# Autodesk Inventor assembly: El Cangrejo
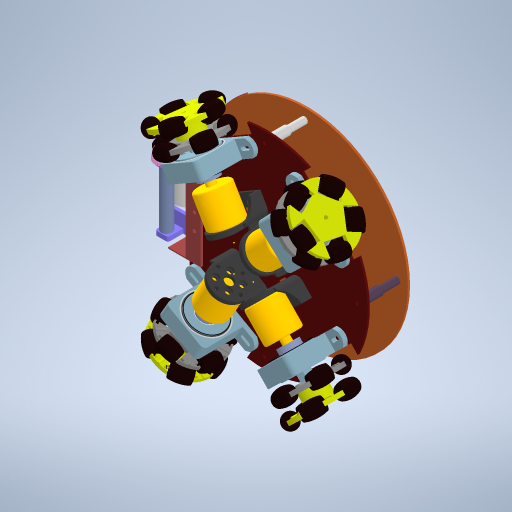
[picture p0: Inventor's stored thumbnail of the model, 512x512]
Saved by Autodesk Inventor 2024.2 (Build 282272000, 272)
## iProperties
Created: 2023-11-20
Part Number: El Cangrejo
Document SubType Name: Assembly
Designer: felip
Author: felip
## Documents named in this file (9)
- C:\Users\felip\Documentos\Robocupp-Mecanica\Gemelo Digital V2\El Cangrejo.iam
- C:\Users\felip\Documentos\Robocupp-Mecanica\Gemelo Digital V2\Motor-Soporte-Montaje.iam
- C:\Users\felip\Documentos\Robocupp-Mecanica\Gemelo Digital V2\Engranaje-Planetario-Montaje.iam
- C:\Users\felip\Documentos\Robocupp-Mecanica\Gemelo Digital V2\BaseV3-Piso2-Step.ipt
- C:\Users\felip\Documentos\Robocupp-Mecanica\Gemelo Digital V2\OMNIWHEELV4.iam
- C:\Users\felip\Documentos\Robocupp-Mecanica\Gemelo Digital V2\Pilar.ipt
- C:\Users\felip\Documentos\Robocupp-Mecanica\Gemelo Digital V2\Part Studio 1 - Part 1.ipt
- C:\Users\felip\Documentos\Robocupp-Mecanica\Gemelo Digital V2\Base-Dribler.ipt
- C:\Users\felip\Documentos\Robocupp-Mecanica\Gemelo Digital V2\Dribler-Desmontable.iam
## Components (19 placed, 8 different names)
1. Motor-Soporte-Montaje:1 [sub-assembly] — Rotational:5, Rotational:6, Cylindrical:4
2. Engranaje-Planetario-Montaje:1 [sub-assembly] — Cylindrical:3, Mate:3, Rotational:18
3. BaseV3-Piso2-Step:1 — Rotational:16, Rotational:17, Rotational:22, Rotational:23
4. OMNIWHEELV4:1 [sub-assembly] — Rotational:18
5. Pilar:1 — Rotational:13
6. Motor-Soporte-Montaje:2 [sub-assembly] — Rotational:7, Rotational:8, Cylindrical:2
7. Motor-Soporte-Montaje:3 [sub-assembly] — Rotational:3, Rotational:4, Cylindrical:1
8. Motor-Soporte-Montaje:4 [sub-assembly] — Rotational:1, Rotational:2, Cylindrical:3
9. Engranaje-Planetario-Montaje:2 [sub-assembly] — Cylindrical:1, Flush:1, Rotational:21
10. Engranaje-Planetario-Montaje:3 [sub-assembly] — Cylindrical:4, Flush:2, Rotational:20
11. Engranaje-Planetario-Montaje:4 [sub-assembly] — Cylindrical:2, Mate:1, Mate:2, Rotational:19
12. OMNIWHEELV4:2 [sub-assembly] — Rotational:19
13. OMNIWHEELV4:3 [sub-assembly] — Rotational:20
14. OMNIWHEELV4:4 [sub-assembly] — Rotational:21
15. Part Studio 1 - Part 1:1 — Rotational:1, Rotational:2, Rotational:3, Rotational:4, Rotational:5, Rotational:6, Rotational:7, Rotational:8, Flush:1, Mate:1, Mate:2, Mate:3, Flush:2, Rotational:13, Rotational:14, Rotational:15
16. Pilar:2 — Rotational:15, Rotational:17
17. Pilar:3 — Rotational:14, Rotational:16
18. Base-Dribler:1 — Rotational:22, Rotational:23, Planar:1, Planar:2
19. Dribler-Desmontable:1 [sub-assembly] — Planar:1, Planar:2
## Relationships (30: RevoluteJoint 19, CylindricalJoint 4, Mate 3, Flush 2, PlanarJoint 2)
- Rotational:1 [RevoluteJoint]: Motor-Soporte-Montaje:4 ↔ Part Studio 1 - Part 1:1
- Rotational:2 [RevoluteJoint]: Motor-Soporte-Montaje:4 ↔ Part Studio 1 - Part 1:1
- Rotational:3 [RevoluteJoint]: Motor-Soporte-Montaje:3 ↔ Part Studio 1 - Part 1:1
- Rotational:4 [RevoluteJoint]: Motor-Soporte-Montaje:3 ↔ Part Studio 1 - Part 1:1
- Rotational:5 [RevoluteJoint]: Motor-Soporte-Montaje:1 ↔ Part Studio 1 - Part 1:1
- Rotational:6 [RevoluteJoint]: Motor-Soporte-Montaje:1 ↔ Part Studio 1 - Part 1:1
- Rotational:7 [RevoluteJoint]: Motor-Soporte-Montaje:2 ↔ Part Studio 1 - Part 1:1
- Rotational:8 [RevoluteJoint]: Motor-Soporte-Montaje:2 ↔ Part Studio 1 - Part 1:1
- Cylindrical:1: Motor-Soporte-Montaje:3 ↔ Engranaje-Planetario-Montaje:2
- Flush:1: Engranaje-Planetario-Montaje:2 ↔ Part Studio 1 - Part 1:1
- Cylindrical:2: Motor-Soporte-Montaje:2 ↔ Engranaje-Planetario-Montaje:4
- Mate:1: Engranaje-Planetario-Montaje:4 ↔ Part Studio 1 - Part 1:1
- Mate:2: Engranaje-Planetario-Montaje:4 ↔ Part Studio 1 - Part 1:1
- Cylindrical:3: Engranaje-Planetario-Montaje:1 ↔ Motor-Soporte-Montaje:4
- Mate:3: Engranaje-Planetario-Montaje:1 ↔ Part Studio 1 - Part 1:1
- Cylindrical:4: Motor-Soporte-Montaje:1 ↔ Engranaje-Planetario-Montaje:3
- Flush:2: Engranaje-Planetario-Montaje:3 ↔ Part Studio 1 - Part 1:1
- Rotational:13 [RevoluteJoint]: Pilar:1 ↔ Part Studio 1 - Part 1:1
- Rotational:14 [RevoluteJoint]: Part Studio 1 - Part 1:1 ↔ Pilar:3
- Rotational:15 [RevoluteJoint]: Part Studio 1 - Part 1:1 ↔ Pilar:2
- Rotational:16 [RevoluteJoint]: BaseV3-Piso2-Step:1 ↔ Pilar:3
- Rotational:17 [RevoluteJoint]: BaseV3-Piso2-Step:1 ↔ Pilar:2
- Rotational:18 [RevoluteJoint]: Engranaje-Planetario-Montaje:1 ↔ OMNIWHEELV4:1
- Rotational:19 [RevoluteJoint]: Engranaje-Planetario-Montaje:4 ↔ OMNIWHEELV4:2
- Rotational:20 [RevoluteJoint]: Engranaje-Planetario-Montaje:3 ↔ OMNIWHEELV4:3
- Rotational:21 [RevoluteJoint]: Engranaje-Planetario-Montaje:2 ↔ OMNIWHEELV4:4
- Rotational:22 [RevoluteJoint]: BaseV3-Piso2-Step:1 ↔ Base-Dribler:1
- Rotational:23 [RevoluteJoint]: BaseV3-Piso2-Step:1 ↔ Base-Dribler:1
- Planar:1: Base-Dribler:1 ↔ Dribler-Desmontable:1
- Planar:2: Base-Dribler:1 ↔ Dribler-Desmontable:1
